# Autodesk Inventor assembly: RECOMPENSA
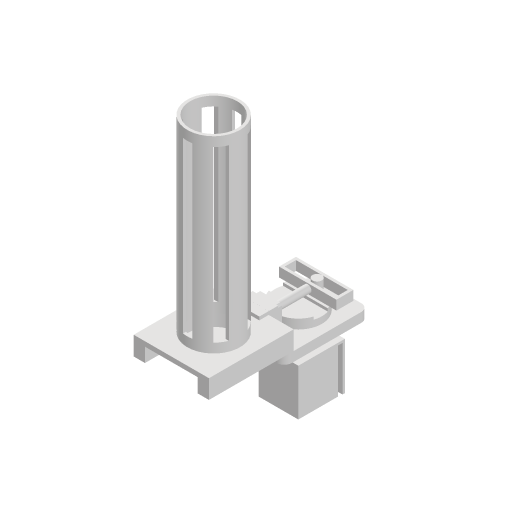
[picture p0: Inventor's stored thumbnail of the model, 512x512]
Saved by Autodesk Inventor 2024 (Build 280153000, 153)
## iProperties
Created: 2024-06-30
Part Number: RECOMPENSA
Document SubType Name: Assembly
Designer: Jhuliams
Author: Jhuliams
## Documents named in this file (9)
- C:\Users\Jhuliams\Documents\GitHub\RECICLADOR_MODELO_3D\MECANISMO DE RECOMPENSA\RECOMPENSA.iam
- C:\Users\Jhuliams\Documents\GitHub\RECICLADOR_MODELO_3D\MECANISMO DE RECOMPENSA\BASE DE YUGO ESCOCES.ipt
- C:\Users\Jhuliams\Documents\GitHub\RECICLADOR_MODELO_3D\MECANISMO DE RECOMPENSA\GUIA GIRATORIA.ipt
- C:\Users\Jhuliams\Documents\GitHub\RECICLADOR_MODELO_3D\MECANISMO DE RECOMPENSA\YUGO.ipt
- C:\Users\Jhuliams\Documents\GitHub\RECICLADOR_MODELO_3D\MECANISMO DE RECOMPENSA\RODAMIENTO LINEAL.ipt
- C:\Users\Jhuliams\Documents\GitHub\RECICLADOR_MODELO_3D\MECANISMO DE RECOMPENSA\PIN.ipt
- C:\Users\Jhuliams\Documents\GitHub\RECICLADOR_MODELO_3D\MECANISMO DE RECOMPENSA\TUBO CONTENEDOR.ipt
- C:\Users\Jhuliams\Documents\GitHub\RECICLADOR_MODELO_3D\MECANISMO DE RECOMPENSA\NEMA 17 PARA TAPA PRINCIPAL.ipt
- C:\Users\Jhuliams\Documents\GitHub\RECICLADOR_MODELO_3D\MECANISMO DE COMPACTADO\SOPORTE DE NEMA.ipt
## Components (8 placed, 8 different names)
1. BASE DE YUGO ESCOCES:1 — Mate:1, Mate:5, Mate:7, Flush:2, Mate:11
2. GUIA GIRATORIA:1 — Mate:1, Mate:8, Mate:9, Mate:12, Mate:14
3. RODAMIENTO LINEAL:1 — Mate:5, Mate:6, Mate:7, Flush:2, Mate:10
4. YUGO:1 — Mate:6, Mate:8, Flush:3, Tangent:1
5. PIN:1 — Mate:9, Flush:3, Tangent:1
6. TUBO CONTENEDOR:1 — Mate:10, Mate:11
7. NEMA 17 PARA TAPA PRINCIPAL:1 — Mate:12, Mate:13, Flush:4
8. SOPORTE DE NEMA:1 — Mate:13, Flush:4, Mate:14
## Relationships (15: Mate 11, Flush 3, Tangent 1)
- Mate:1: BASE DE YUGO ESCOCES:1 ↔ GUIA GIRATORIA:1
- Mate:5: BASE DE YUGO ESCOCES:1 ↔ RODAMIENTO LINEAL:1
- Mate:6: RODAMIENTO LINEAL:1 ↔ YUGO:1
- Mate:7: BASE DE YUGO ESCOCES:1 ↔ RODAMIENTO LINEAL:1
- Flush:2 (1 mm): BASE DE YUGO ESCOCES:1 ↔ RODAMIENTO LINEAL:1
- Mate:8: GUIA GIRATORIA:1 ↔ YUGO:1
- Mate:9: GUIA GIRATORIA:1 ↔ PIN:1
- Flush:3: YUGO:1 ↔ PIN:1
- Tangent:1: YUGO:1 ↔ PIN:1
- Mate:10: RODAMIENTO LINEAL:1 ↔ TUBO CONTENEDOR:1
- Mate:11: BASE DE YUGO ESCOCES:1 ↔ TUBO CONTENEDOR:1
- Mate:12: GUIA GIRATORIA:1 ↔ NEMA 17 PARA TAPA PRINCIPAL:1
- Mate:13: NEMA 17 PARA TAPA PRINCIPAL:1 ↔ SOPORTE DE NEMA:1
- Flush:4: NEMA 17 PARA TAPA PRINCIPAL:1 ↔ SOPORTE DE NEMA:1
- Mate:14 (5 mm): GUIA GIRATORIA:1 ↔ SOPORTE DE NEMA:1
